# Autodesk Inventor assembly: 22nc_plate5_motor_nomo_12580
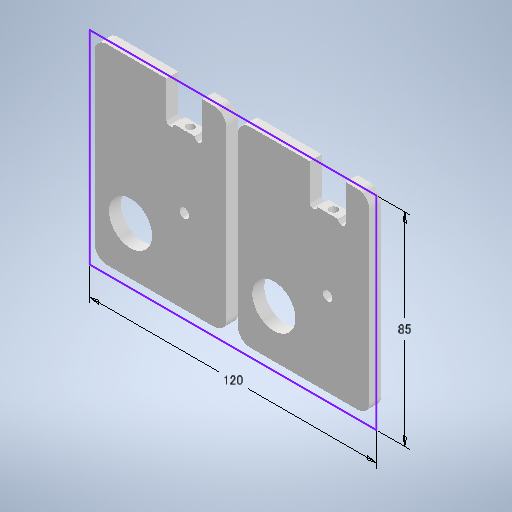
[picture p0: Inventor's stored thumbnail of the model, 512x512]
Saved by Autodesk Inventor 2025.1 (Build 291241000, 241)
## iProperties
Created: 2025-05-06
Part Number: 22nc_plate5_motor_nomo_12580
Document SubType Name: Assembly
Designer: yuki0520
Author: yuki0520
## Documents named in this file (2)
- C:\Users\yuki0520\OneDrive\ドキュメント\Inventor\2025_nhk\tanaka\nageru\light\22nc_plate5_motor_nomo_12580.iam
- C:\Users\yuki0520\OneDrive\ドキュメント\Inventor\2025_nhk\tanaka\nageru\light\light_plate_nomo.ipt
## Components (2 placed, 1 different names)
1. light_plate_nomo:1 — メイト:1, フラッシュ:1, フラッシュ:2
2. light_plate_nomo:2 — メイト:1, フラッシュ:1, フラッシュ:2
## Relationships (3: Flush 2, Mate 1)
- メイト:1 [Mate] (5 mm): light_plate_nomo:1 ↔ light_plate_nomo:2
- フラッシュ:1 [Flush]: light_plate_nomo:1 ↔ light_plate_nomo:2
- フラッシュ:2 [Flush]: light_plate_nomo:1 ↔ light_plate_nomo:2
